# Autodesk Inventor assembly: Stromversorgung
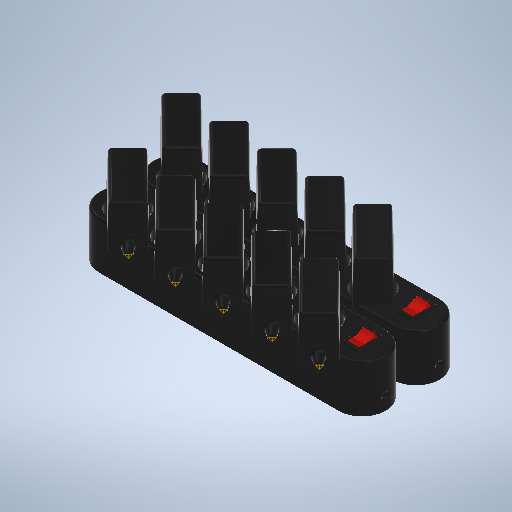
[picture p0: Inventor's stored thumbnail of the model, 512x512]
Saved by Autodesk Inventor 2025.1 (Build 291241000, 241)
## iProperties
Created: 2024-11-07
Part Number: Stromversorgung
Document SubType Name: Assembly
Designer: Kai Altwicker
Author: Kai Altwicker
## iProperties of the stored document Rocker.prt.ipt
Created: 2019-03-21
Part Number: Rocker.prt
Material: Generisch
Document SubType Name: Modeling
Designer: Kai Altwicker
Density: 1 g/cm^3
Appearance: Vorgabe
Author: Kai Altwicker
Revision Number: TUTTO
## iProperties of the stored document Terminal.prt.ipt
Created: 2019-03-21
Part Number: Terminal.prt
Material: Generisch
Document SubType Name: Modeling
Designer: Kai Altwicker
Density: 1 g/cm^3
Appearance: Vorgabe
Author: Kai Altwicker
Revision Number: TUTTO
## iProperties of the stored document ARCOLECTRIC_H8600VB.prt.iam
Created: 2019-03-21
Part Number: ARCOLECTRIC_H8600VB.prt
Document SubType Name: Assembly
Designer: Kai Altwicker
Author: Kai Altwicker
Revision Number: TUTTO
## iProperties of the stored document Housing.prt.ipt
Created: 2019-03-21
Part Number: Housing.prt
Material: Generisch
Document SubType Name: Modeling
Designer: Kai Altwicker
Density: 1 g/cm^3
Appearance: Vorgabe
Author: Kai Altwicker
Revision Number: TUTTO
## iProperties of the stored document ciabatta.ipt
Created: 2019-03-21
Part Number: ciabatta
Material: Generisch
Document SubType Name: Modeling
Designer: Kai Altwicker
Density: 1 g/cm^3
Appearance: Vorgabe
Author: Kai Altwicker
Revision Number: TUTTO
## iProperties of the stored document Assieme1_ciabatta_interrutore_.iam
Created: 2019-03-21
Part Number: Assieme1_ciabatta_interrutore_
Description: STEP AP203
Document SubType Name: Assembly
Designer: Kai Altwicker
Sending System: SolidWorks 2019
Preprocessor: SwSTEP 2.0
Title: Assieme1_ciabatta_interrutore_.STEP
Revision Number: TUTTO
## Documents named in this file (11)
- C:\Users\tallA\Repos\VolumanXR\hardware-capture\cad\rig_v2\Stromversorgung.iam
- **C:\Users\tallA\Repos\VolumanXR\hardware-capture\cad\rig_v2\Stromversorgung.iam*LocalDocs*xAaaaqpcaAaaaaaaaAaaaahe1Ig*Assieme1_ciabatta_interrutore_.iam
- C:\Users\tallA\Repos\VolumanXR\hardware-capture\cad\Library\Netzteil.ipt
- **C:\Users\tallA\Repos\VolumanXR\hardware-capture\cad\rig_v2\Rig_v2\Stromversorgung.iam*LocalDocs*xAaaaascaAaaaaaaaAaaaaftiRg*Rocker.prt.ipt
- **C:\Users\tallA\Repos\VolumanXR\hardware-capture\cad\rig_v2\Rig_v2\Stromversorgung.iam*LocalDocs*xAaaaa1daAaaaaaaaAaaaq0p5He*Terminal.prt.ipt
- **C:\Users\tallA\Repos\VolumanXR\hardware-capture\cad\rig_v2\Rig_v2\Stromversorgung.iam*LocalDocs*xAaaaazdaAaaaaaaaAaaaasm55c*ARCOLECTRIC_H8600VB.prt.iam
- **C:\Users\tallA\Repos\VolumanXR\hardware-capture\cad\rig_v2\Rig_v2\Stromversorgung.iam*LocalDocs*xAaaaayaaAaaaaaaaAaaaqjzlEe*Housing.prt.ipt
- **C:\Users\tallA\Repos\VolumanXR\hardware-capture\cad\rig_v2\Rig_v2\Stromversorgung.iam*LocalDocs*xAaaaq2daAaaaaaaaAaaaa3dhUg*ciabatta.ipt
- **C:\Users\tallA\Repos\VolumanXR\hardware-capture\cad\rig_v2\Rig_v2\Stromversorgung.iam*LocalDocs*xAaaaqpcaAaaaaaaaAaaaahe1Ig*Assieme1_ciabatta_interrutore_.iam
- C:\Users\tallA\Repos\VolumanXR\hardware-capture\cad\dimensions.xlsx
- C:\Users\tallA\Repos\VolumanXR\hardware-capture\cad\Library\Assieme1_ciabatta_interrutore_.STEP
## Components (12 placed, 2 different names)
1. Assieme1_ciabatta_interrutore_:1 [sub-assembly] — Fluchtend:1, Fluchtend:2, Passend:1, Passend:13, Passend:14, Passend:15, Passend:16, Passend:17, Passend:18, Passend:19, Passend:20, Passend:21, Passend:22, Passend:23
2. Assieme1_ciabatta_interrutore_:2 [sub-assembly] — Fluchtend:1, Fluchtend:2, Passend:1, Passend:2, Passend:3, Passend:4, Passend:5, Passend:6, Passend:7, Passend:8, Passend:9, Passend:10, Passend:11, Passend:12
3. Netzteil:1 — Fluchtend:3, Passend:2, Passend:3
4. Netzteil:2 — Fluchtend:3, Fluchtend:4, Passend:4, Passend:5
5. Netzteil:3 — Fluchtend:4, Fluchtend:10, Passend:6, Passend:7
6. Netzteil:4 — Fluchtend:5, Fluchtend:10, Passend:8, Passend:9
7. Netzteil:5 — Fluchtend:5, Passend:10, Passend:11, Passend:12
8. Netzteil:6 — Fluchtend:9, Passend:15, Passend:16
9. Netzteil:7 — Fluchtend:8, Fluchtend:9, Passend:13, Passend:14, Passend:23
10. Netzteil:8 — Fluchtend:7, Fluchtend:8, Passend:17, Passend:18
11. Netzteil:9 — Fluchtend:6, Fluchtend:7, Passend:19, Passend:20
12. Netzteil:10 — Fluchtend:6, Passend:21, Passend:22
## Relationships (33: Mate 23, Flush 10)
- Fluchtend:1 [Flush]: Assieme1_ciabatta_interrutore_:1 ↔ Assieme1_ciabatta_interrutore_:2
- Fluchtend:2 [Flush]: Assieme1_ciabatta_interrutore_:1 ↔ Assieme1_ciabatta_interrutore_:2
- Passend:1 [Mate] (5 mm): Assieme1_ciabatta_interrutore_:1 ↔ Assieme1_ciabatta_interrutore_:2
- Fluchtend:3 [Flush]: Netzteil:1 ↔ Netzteil:2
- Fluchtend:4 [Flush]: Netzteil:2 ↔ Netzteil:3
- Fluchtend:5 [Flush]: Netzteil:4 ↔ Netzteil:5
- Fluchtend:6 [Flush]: Netzteil:9 ↔ Netzteil:10
- Fluchtend:7 [Flush]: Netzteil:8 ↔ Netzteil:9
- Fluchtend:8 [Flush]: Netzteil:7 ↔ Netzteil:8
- Fluchtend:9 [Flush]: Netzteil:6 ↔ Netzteil:7
- Fluchtend:10 [Flush]: Netzteil:3 ↔ Netzteil:4
- Passend:2 [Mate]: Assieme1_ciabatta_interrutore_:2 ↔ Netzteil:1
- Passend:3 [Mate] (0.1 mm): Assieme1_ciabatta_interrutore_:2 ↔ Netzteil:1
- Passend:4 [Mate]: Assieme1_ciabatta_interrutore_:2 ↔ Netzteil:2
- Passend:5 [Mate] (0.1 mm): Assieme1_ciabatta_interrutore_:2 ↔ Netzteil:2
- Passend:6 [Mate]: Assieme1_ciabatta_interrutore_:2 ↔ Netzteil:3
- Passend:7 [Mate] (0.1 mm): Assieme1_ciabatta_interrutore_:2 ↔ Netzteil:3
- Passend:8 [Mate]: Assieme1_ciabatta_interrutore_:2 ↔ Netzteil:4
- Passend:9 [Mate] (0.1 mm): Assieme1_ciabatta_interrutore_:2 ↔ Netzteil:4
- Passend:10 [Mate]: Assieme1_ciabatta_interrutore_:2 ↔ Netzteil:5
- Passend:11 [Mate] (0.1 mm): Assieme1_ciabatta_interrutore_:2 ↔ Netzteil:5
- Passend:12 [Mate]: Assieme1_ciabatta_interrutore_:2 ↔ Netzteil:5
- Passend:13 [Mate]: Assieme1_ciabatta_interrutore_:1 ↔ Netzteil:7
- Passend:14 [Mate] (0.1 mm): Assieme1_ciabatta_interrutore_:1 ↔ Netzteil:7
- Passend:15 [Mate]: Assieme1_ciabatta_interrutore_:1 ↔ Netzteil:6
- Passend:16 [Mate] (0.1 mm): Assieme1_ciabatta_interrutore_:1 ↔ Netzteil:6
- Passend:17 [Mate]: Assieme1_ciabatta_interrutore_:1 ↔ Netzteil:8
- Passend:18 [Mate] (0.1 mm): Assieme1_ciabatta_interrutore_:1 ↔ Netzteil:8
- Passend:19 [Mate]: Assieme1_ciabatta_interrutore_:1 ↔ Netzteil:9
- Passend:20 [Mate] (0.1 mm): Assieme1_ciabatta_interrutore_:1 ↔ Netzteil:9
- Passend:21 [Mate]: Assieme1_ciabatta_interrutore_:1 ↔ Netzteil:10
- Passend:22 [Mate] (0.1 mm): Assieme1_ciabatta_interrutore_:1 ↔ Netzteil:10
- Passend:23 [Mate]: Assieme1_ciabatta_interrutore_:1 ↔ Netzteil:7
## Named parameters: d_tol = 0.3 mm, d_wand = 1.5 mm, l_profil_traeger = 1500 mm, l_profil_staender = 2500 mm, b_profil_40x40 = 40 mm, b_profil_20x20 = 20 mm, h_profil_20x20 = 20 mm, h_profil_40x40 = 40 mm, l_profil_40x40 = 2500 mm, d_traeger = 625 mm, l_profil_20x20 = 1500 mm, b_rasp_pi = 56 mm, l_rasp_pi = 85 mm, D_hexadeca = 7541.00924 mm, D_oct = 3621.32034 mm, w_kamera_hori = 66 deg, w_kamera_vert = 41 deg, r_rasp_pi = 3 mm
